# Autodesk Inventor assembly: Frame
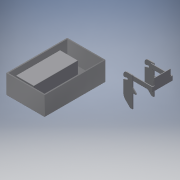
[picture p0: Inventor's stored thumbnail of the model, 180x180]
Saved by Autodesk Inventor 2018 (Build 220112000, 112)
## iProperties
Created: 2018-08-10
Part Number: Frame
Document SubType Name: Assembly
Designer: ruben
Author: ruben
## Documents named in this file (5)
- C:\Users\ruben\Documents\Inventor\Electric-Scooter\Frame\Frame.iam
- C:\Users\ruben\Documents\Inventor\Electric-Scooter\Frame\Rear Wheel Holder.ipt
- C:\Users\ruben\Documents\Inventor\Electric-Scooter\Frame\Footboard - feet protect holder.ipt
- C:\Users\ruben\Documents\Inventor\Electric-Scooter\Frame\Batterybox 2\Batterybox 2.ipt
- C:\Users\ruben\Documents\Inventor\Electric-Scooter\Frame\Batterybox 2\Waterproof box 2.ipt
## Components (5 placed, 4 different names)
1. Rear Wheel Holder:1 — Mate:4, Flush:1, Flush:2, Flush:3, Flush:4
2. Rear Wheel Holder:2 — Mate:5, Flush:3, Flush:4
3. Footboard - feet protect holder:1 — Mate:4, Flush:1, Flush:2, Mate:5
4. Batterybox 2:1 — Mate:1, Mate:2, Mate:3
5. Waterproof box 2:1 — Mate:1, Mate:2, Mate:3
## Relationships (9: Mate 5, Flush 4)
- Mate:1: Batterybox 2:1 ↔ Waterproof box 2:1
- Mate:2 (32.5 mm): Batterybox 2:1 ↔ Waterproof box 2:1
- Mate:3 (1 mm): Batterybox 2:1 ↔ Waterproof box 2:1
- Mate:4: Rear Wheel Holder:1 ↔ Footboard - feet protect holder:1
- Flush:1 (85 mm): Rear Wheel Holder:1 ↔ Footboard - feet protect holder:1
- Flush:2 (-4 mm): Rear Wheel Holder:1 ↔ Footboard - feet protect holder:1
- Mate:5: Rear Wheel Holder:2 ↔ Footboard - feet protect holder:1
- Flush:3: Rear Wheel Holder:1 ↔ Rear Wheel Holder:2
- Flush:4: Rear Wheel Holder:1 ↔ Rear Wheel Holder:2
